# Autodesk Inventor assembly: Wheel
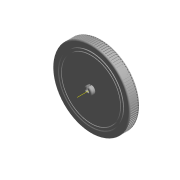
[picture p0: Inventor's stored thumbnail of the model, 180x180]
Saved by Autodesk Inventor 2014 (Build 180170000, 170)
## iProperties
Created: 2013-06-25
Part Number: Wheel
Document SubType Name: Assembly
Designer: Felix
Author: Felix
## Documents named in this file (4)
- C:\Users\Felix\Desktop\Beep\Hardware\3D-CAD\parts\Pololu_Wheel_6mm\Wheel.iam
- C:\Users\Felix\Desktop\Beep\Hardware\3D-CAD\parts\Pololu_Wheel_6mm\felloe.ipt
- C:\Users\Felix\Desktop\Beep\Hardware\3D-CAD\parts\Pololu_Wheel_6mm\tire.ipt
- C:\Users\Felix\Desktop\Beep\Hardware\3D-CAD\encoder_wheel.ipt
## Components (3 placed, 3 different names)
1. felloe:1 — Passend:1, Passend:2, Fluchtend:1, Passend:3, Passend:4, Fluchtend:2
2. tire:1 — Passend:1, Fluchtend:1
3. encoder_wheel:1 — Fluchtend:2
## Relationships (6: Mate 4, Flush 2)
- Passend:1 [Mate]: felloe:1 ↔ tire:1
- Passend:2 [Mate]: felloe:1
- Fluchtend:1 [Flush]: felloe:1 ↔ tire:1
- Passend:3 [Mate]: felloe:1
- Passend:4 [Mate]: felloe:1
- Fluchtend:2 [Flush]: felloe:1 ↔ encoder_wheel:1
